# Autodesk Inventor assembly: Assembly1
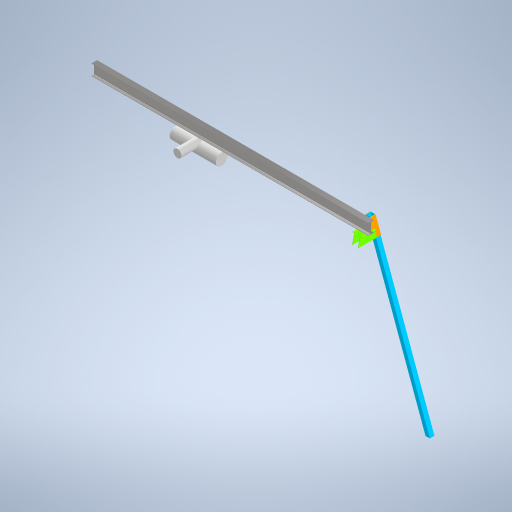
[picture p0: Inventor's stored thumbnail of the model, 512x512]
Saved by Autodesk Inventor 2024.2 (Build 282272000, 272)
## iProperties
Created: 2024-06-11
Part Number: Assembly1
Document SubType Name: Assembly
Designer: admin
Author: admin
## Documents named in this file (9)
- C:\Users\admin\YandexDisk-badmisterfox\домашниий пк\Inventor\Workshop\оборудование\Кран козловой 2\Assembly1.iam
- C:\Users\admin\YandexDisk-badmisterfox\домашниий пк\Inventor\Workshop\оборудование\Двутавр 240x36 - 6000.ipt
- C:\Users\admin\YandexDisk-badmisterfox\домашниий пк\Inventor\Workshop\оборудование\Кран козловой 2\WRS 000,000 кран козловой 6х4.ipt
- C:\Users\admin\YandexDisk-badmisterfox\домашниий пк\Inventor\Workshop\оборудование\Кран козловой 2\Тельфер Таль электрическая.ipt
- C:\Users\admin\YandexDisk-badmisterfox\домашниий пк\Inventor\Workshop\оборудование\Кран козловой 2\полка под швеллер.ipt
- C:\Users\admin\YandexDisk-badmisterfox\домашниий пк\Inventor\Workshop\оборудование\Кран козловой 2\стойка 1 100x100x4 - 5000.ipt
- C:\Users\admin\YandexDisk-badmisterfox\домашниий пк\Inventor\Workshop\оборудование\Кран козловой 2\держатель полки 1.ipt
- C:\Users\admin\YandexDisk-badmisterfox\домашниий пк\Inventor\Workshop\оборудование\Кран козловой 2\Ухо на швеллер пямое.ipt
- C:\Users\admin\YandexDisk-badmisterfox\домашниий пк\Inventor\Workshop\оборудование\Кран козловой 2\Ухо на стойку.ipt
## Components (11 placed, 8 different names)
1. Двутавр 240x36 - 6000:1 — Flush:1, Mate:1, Flush:2, Flush:4, Mate:5, Mate:7, Mate:11, Mate:12, Mate:14
2. WRS 000,000 кран козловой 6х4:1 — Mate:2, Mate:3, Flush:3
3. Тельфер Таль электрическая:1 — Flush:4, Mate:4
4. полка под швеллер:1 — Mate:5, Flush:8, Rigid:4
5. стойка 1 100x100x4 - 5000:1 — Flush:11, Mate:8, Flush:12, Mate:9, Flush:13, Flush:14, Mate:10, Flush:15, Flush:16
6. держатель полки 1:2 — Rigid:4, Mate:9, Flush:13, Flush:14
7. Ухо на швеллер пямое:1 — Mate:7, Flush:11, Mate:11
8. Ухо на стойку:1 — Mate:8, Flush:12
9. полка под швеллер:2 — Rigid:5
10. держатель полки 1:3 — Mate:10, Flush:15, Flush:16, Rigid:5, Mate:13
11. Ухо на швеллер пямое:2 — Mate:12, Mate:13, Mate:14
## Relationships (26: Mate 13, Flush 11, WeldJoint 2)
- Flush:1 (4850 mm): Двутавр 240x36 - 6000:1
- Mate:1: Двутавр 240x36 - 6000:1
- Flush:2: Двутавр 240x36 - 6000:1
- Mate:2: WRS 000,000 кран козловой 6х4:1
- Mate:3: WRS 000,000 кран козловой 6х4:1
- Flush:3: WRS 000,000 кран козловой 6х4:1
- Flush:4: Двутавр 240x36 - 6000:1 ↔ Тельфер Таль электрическая:1
- Mate:4: Тельфер Таль электрическая:1
- Mate:5: Двутавр 240x36 - 6000:1 ↔ полка под швеллер:1
- Flush:8: полка под швеллер:1
- Mate:7: Двутавр 240x36 - 6000:1 ↔ Ухо на швеллер пямое:1
- Flush:11: стойка 1 100x100x4 - 5000:1 ↔ Ухо на швеллер пямое:1
- Mate:8: стойка 1 100x100x4 - 5000:1 ↔ Ухо на стойку:1
- Flush:12: стойка 1 100x100x4 - 5000:1 ↔ Ухо на стойку:1
- Rigid:4 [WeldJoint]: полка под швеллер:1 ↔ держатель полки 1:2
- Mate:9: стойка 1 100x100x4 - 5000:1 ↔ держатель полки 1:2
- Flush:13: стойка 1 100x100x4 - 5000:1 ↔ держатель полки 1:2
- Flush:14: стойка 1 100x100x4 - 5000:1 ↔ держатель полки 1:2
- Mate:10: стойка 1 100x100x4 - 5000:1 ↔ держатель полки 1:3
- Flush:15: стойка 1 100x100x4 - 5000:1 ↔ держатель полки 1:3
- Flush:16: стойка 1 100x100x4 - 5000:1 ↔ держатель полки 1:3
- Mate:11: Двутавр 240x36 - 6000:1 ↔ Ухо на швеллер пямое:1
- Rigid:5 [WeldJoint]: полка под швеллер:2 ↔ держатель полки 1:3
- Mate:12: Двутавр 240x36 - 6000:1 ↔ Ухо на швеллер пямое:2
- Mate:13: держатель полки 1:3 ↔ Ухо на швеллер пямое:2
- Mate:14: Двутавр 240x36 - 6000:1 ↔ Ухо на швеллер пямое:2
